# Autodesk Inventor assembly: bearing block outer
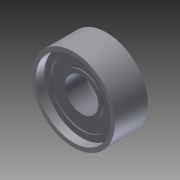
[picture p0: Inventor's stored thumbnail of the model, 180x180]
Saved by Autodesk Inventor 2012 (Build 160160000, 160)
## iProperties
Created: 2012-02-07
Part Number: bearing block outer
Document SubType Name: Assembly
Designer: Antonella Wilby
Author: Antonella Wilby
## Documents named in this file (3)
- C:\Users\Antonella\Documents\GCC Robotics 2012 - Mechanical\Robot 2.0\Drive Train\bearing block outer.iam
- C:\Users\Antonella\Documents\GCC Robotics 2012 - Mechanical\Robot 2.0\Drive Train\bearing block outer.ipt
- C:\Users\Antonella\Documents\GCC Robotics 2012 - Mechanical\Robot 2.0\Drive Train\R8-ZZ.ipt
## Components (2 placed, 2 different names)
1. bearing block outer:1 — Mate:1, Mate:2
2. R8-ZZ:1 — Mate:1, Mate:2
## Relationships (2: Mate 2)
- Mate:1: bearing block outer:1 ↔ R8-ZZ:1
- Mate:2: bearing block outer:1 ↔ R8-ZZ:1
